# Autodesk Inventor assembly: ROBUSTAv2
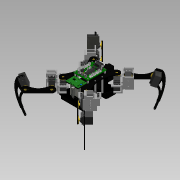
[picture p0: Inventor's stored thumbnail of the model, 180x180]
Saved by Autodesk Inventor 2015 SP1 (Build 190203100, 203)
## iProperties
Created: 2015-01-25
Part Number: ROBUSTAv2
Document SubType Name: Assembly
Designer: Rafi Kurnia Putra
Author: Rafi Kurnia Putra
## Documents named in this file (19)
- D:\Dropbox\krpai berkaki trui 2015\ROBUSTA\MEKANIK\ROBUSTA\Assembly Base.iam
- D:\Dropbox\krpai berkaki trui 2015\ROBUSTA\MEKANIK\ROBUSTA\Base Bawah V2.ipt
- D:\Dropbox\krpai berkaki trui 2015\ROBUSTA\MEKANIK\ROBUSTA\Base Atas V2.ipt
- D:\Dropbox\krpai berkaki trui 2015\ROBUSTA\MEKANIK\ROBUSTA\Spacer 5cm.ipt
- D:\Dropbox\krpai berkaki trui 2015\ROBUSTA\MEKANIK\ROBUSTA\Cover UBEC.ipt
- D:\Dropbox\krpai berkaki trui 2015\ROBUSTA\MEKANIK\ROBUSTA\ssc-32.ipt
- D:\Dropbox\krpai berkaki trui 2015\ROBUSTA\MEKANIK\ROBUSTA\Spacer 1cm.ipt
- D:\Dropbox\krpai berkaki trui 2015\ROBUSTA\MEKANIK\ROBUSTA\servo.ipt
- D:\Dropbox\krpai berkaki trui 2015\ROBUSTA\MEKANIK\ROBUSTA\Horn Servo.ipt
- D:\Dropbox\krpai berkaki trui 2015\ROBUSTA\MEKANIK\ROBUSTA\Femur.ipt
- D:\Dropbox\krpai berkaki trui 2015\ROBUSTA\MEKANIK\ROBUSTA\Bearing Besar.ipt
- D:\Dropbox\krpai berkaki trui 2015\ROBUSTA\MEKANIK\ROBUSTA\Assembly UVTRON.iam
- D:\Dropbox\krpai berkaki trui 2015\ROBUSTA\MEKANIK\ROBUSTA\UVTRON Wall.ipt
- D:\Dropbox\krpai berkaki trui 2015\ROBUSTA\MEKANIK\ROBUSTA\Cover Color Sensor V2.ipt
- D:\Dropbox\krpai berkaki trui 2015\ROBUSTA\MEKANIK\ROBUSTA\2-56 X 0.250 PHS (PHS-02).ipt
- D:\Dropbox\krpai berkaki trui 2015\ROBUSTA\MEKANIK\ROBUSTA\tibia.ipt
- D:\Dropbox\krpai berkaki trui 2015\ROBUSTA\MEKANIK\ROBUSTA\Baterai.ipt
- D:\Dropbox\krpai berkaki trui 2015\ROBUSTA\MEKANIK\ROBUSTA\Braket Servo 2.ipt
- D:\Dropbox\krpai berkaki trui 2015\ROBUSTA\MEKANIK\ROBUSTA\Bracket3.ipt
## Components (67 placed, 18 different names)
1. Base Bawah V2:1 — Mate:1, Mate:2, Mate:3, Mate:4, Mate:5, Mate:6, Mate:7, Mate:8, Mate:13, Mate:14, Mate:15, Mate:169, Mate:170, Mate:171, Mate:203, Mate:204, Mate:205, Mate:311, Angle:18, Flush:2, Flush:3, Angle:19
2. Spacer 5cm:1 — Mate:1, Mate:2, Mate:175, Mate:184, Angle:15, Angle:17, Mate:312
3. Spacer 5cm:2 — Mate:3, Mate:4, Mate:174, Mate:185, Angle:16
4. Spacer 5cm:3 — Mate:5, Mate:6, Mate:172, Angle:16
5. Spacer 5cm:4 — Mate:7, Mate:8, Mate:173, Angle:15
6. Cover UBEC:1 — Mate:13, Mate:14, Mate:15, Insert:7, Insert:8, Mate:314
7. Spacer 1cm:1 — Insert:4, Mate:183, Mate:186
8. Spacer 1cm:2 — Insert:3, Mate:180, Mate:187
9. Spacer 1cm:3 — Mate:181, Mate:188
10. Spacer 1cm:4 — Mate:182, Mate:189
11. ssc-32:1 — Insert:3, Insert:4
12. servo:1 — Mate:28, Mate:29, Mate:290, Mate:291, Mate:292, Angle:13
13. Horn Servo:1 — Mate:28, Mate:29, Mate:152, Mate:153
14. Braket Servo 2:1 — Mate:34, Mate:35, Mate:37, Mate:38, Mate:39, Mate:315, Mate:317
15. Braket Servo 2:2 — Mate:34, Mate:35, Mate:45, Mate:46, Mate:47, Mate:141, Angle:19, Mate:315, Mate:316, Angle:20
16. servo:2 — Mate:37, Mate:38, Mate:39, Mate:40, Mate:41, Mate:42, Mate:318, Mate:319
17. Horn Servo:3 — Mate:40, Mate:41, Mate:42, Mate:150, Mate:151
18. servo:3 — Mate:45, Mate:46, Mate:47, Mate:48, Mate:49
19. Horn Servo:4 — Mate:48, Mate:49, Mate:193, Mate:194
20. servo:4 — Mate:296, Mate:297, Mate:298, Angle:9
21. Horn Servo:5 — Mate:160, Mate:161
22. Braket Servo 2:5 — Mate:325, Mate:327
23. Braket Servo 2:6 — Mate:145, Mate:325, Mate:326, Angle:22
24. servo:5 — Mate:328, Mate:329
25. Horn Servo:6 — Mate:158, Mate:159
26. servo:6 — Angle:7
27. Horn Servo:7 — Mate:191, Mate:196
28. servo:7 — Mate:80, Mate:81, Mate:293, Mate:294, Mate:295, Angle:6
29. Horn Servo:8 — Mate:80, Mate:81, Mate:156, Mate:157
30. Braket Servo 2:4 — Mate:84, Mate:85, Mate:86, Mate:87, Mate:143, Mate:304, Mate:305, 90, Mate:320, Mate:321, Angle:21
31. Braket Servo 2:3 — Mate:84, Mate:85, Mate:86, Mate:92, Mate:93, Mate:94, Mate:320, Mate:322, Mate:323, Mate:324
32. servo:8 — Mate:87, Mate:90, Mate:91, Mate:304, Mate:305
33. Horn Servo:9 — Mate:90, Mate:91, Mate:192, Mate:197
34. servo:9 — Mate:92, Mate:93, Mate:94, Mate:95, Mate:96
35. Horn Servo:10 — Mate:95, Mate:96, Mate:154, Mate:155
36. servo:10 — Mate:299, Mate:300, Mate:301, Angle:12
37. Horn Servo:11 — Mate:164, Mate:165
38. Braket Servo 2:8 — Mate:147, Angle:10, Mate:330, Mate:331, Angle:23
39. Braket Servo 2:7 — Mate:330
40. servo:11
41. Horn Servo:12 — Mate:190, Mate:195
42. servo:12
43. Horn Servo:13 — Mate:162, Mate:163
44. Bearing Besar:1 — Mate:141, Mate:316
45. Bearing Besar:2 — Mate:143, Mate:321
46. Bearing Besar:3 — Mate:145, Mate:326
47. Bearing Besar:4 — Mate:147, Mate:331
48. Femur:1 — Mate:150, Mate:151, Mate:152, Mate:153, Angle:13, Angle:20
49. Femur:2 — Mate:154, Mate:155, Mate:156, Mate:157, Angle:6, Angle:21
50. Femur:3 — Mate:158, Mate:159, Mate:160, Mate:161, Angle:9, Angle:22
51. Femur:4 — Mate:162, Mate:163, Mate:164, Mate:165, Angle:12, Angle:23
52. UVTRON Wall:1 — Mate:169, Mate:170, Mate:171, Tangent:1
53. Base Atas V2:1 — Mate:172, Mate:173, Mate:174, Mate:175, Mate:180, Mate:181, Mate:182, Mate:183, Mate:184, Mate:185, Mate:186, Mate:187, Mate:188, Mate:189, Mate:190, Mate:191, Mate:192, Mate:193, Mate:194, Mate:195, Mate:196, Mate:197, 90, Angle:7, Angle:10, Mate:306, Mate:307, Mate:308, Mate:309, Mate:310
54. Cover Color Sensor V2:1 — Mate:203, Mate:204, Mate:205, Insert:5, Insert:6
55. 2-56 X 0.250 PHS (PHS-02):1 — Insert:6
56. 2-56 X 0.250 PHS (PHS-02):2 — Insert:5
57. 2-56 X 0.250 PHS (PHS-02):3 — Insert:7
58. 2-56 X 0.250 PHS (PHS-02):4 — Insert:8
59. tibia:1 — Mate:290, Mate:291, Mate:292
60. tibia:2 — Mate:296, Mate:297, Mate:298
61. tibia:3 — Mate:299, Mate:300, Mate:301
62. tibia:4 — Mate:293, Mate:294, Mate:295
63. Assembly UVTRON:1 [sub-assembly] — Mate:306, Mate:307, Mate:308, Mate:309, Mate:310
64. Baterai:1 — Mate:311, Angle:17, Mate:312, Tangent:1, Angle:18
65. Bracket3:1 — Mate:317, Mate:318, Mate:319
66. Bracket3:2 — Mate:322, Mate:323, Mate:324
67. Bracket3:3 — Mate:327, Mate:328, Mate:329
## Relationships (180: Mate 155, Angle 16, Insert 6, Flush 2, Tangent 1)
- Mate:1: Base Bawah V2:1 ↔ Spacer 5cm:1
- Mate:2: Base Bawah V2:1 ↔ Spacer 5cm:1
- Mate:3: Base Bawah V2:1 ↔ Spacer 5cm:2
- Mate:4: Base Bawah V2:1 ↔ Spacer 5cm:2
- Mate:5: Base Bawah V2:1 ↔ Spacer 5cm:3
- Mate:6: Base Bawah V2:1 ↔ Spacer 5cm:3
- Mate:7: Base Bawah V2:1 ↔ Spacer 5cm:4
- Mate:8: Base Bawah V2:1 ↔ Spacer 5cm:4
- Mate:13: Base Bawah V2:1 ↔ Cover UBEC:1
- Mate:14: Base Bawah V2:1 ↔ Cover UBEC:1
- Mate:15: Base Bawah V2:1 ↔ Cover UBEC:1
- Insert:3: Spacer 1cm:2 ↔ ssc-32:1
- Insert:4: Spacer 1cm:1 ↔ ssc-32:1
- Mate:28: servo:1 ↔ Horn Servo:1
- Mate:29: servo:1 ↔ Horn Servo:1
- Mate:34: Braket Servo 2:1 ↔ Braket Servo 2:2
- Mate:35: Braket Servo 2:1 ↔ Braket Servo 2:2
- Mate:37: Braket Servo 2:1 ↔ servo:2
- Mate:38: Braket Servo 2:1 ↔ servo:2
- Mate:39: Braket Servo 2:1 ↔ servo:2
- Mate:40: servo:2 ↔ Horn Servo:3
- Mate:41: servo:2 ↔ Horn Servo:3
- Mate:42: servo:2 ↔ Horn Servo:3
- Mate:45: Braket Servo 2:2 ↔ servo:3
- Mate:46: Braket Servo 2:2 ↔ servo:3
- Mate:47: Braket Servo 2:2 ↔ servo:3
- Mate:48: servo:3 ↔ Horn Servo:4
- Mate:49: servo:3 ↔ Horn Servo:4
- [Mate]: servo:4 ↔ Horn Servo:5
- [Mate]: servo:4 ↔ Horn Servo:5
- [Mate]: Braket Servo 2:5 ↔ Braket Servo 2:6
- [Mate]: Braket Servo 2:5 ↔ Braket Servo 2:6
- [Mate]: Braket Servo 2:5 ↔ servo:5
- [Mate]: Braket Servo 2:5 ↔ servo:5
- [Mate]: Braket Servo 2:5 ↔ servo:5
- [Mate]: servo:5 ↔ Horn Servo:6
- [Mate]: servo:5 ↔ Horn Servo:6
- [Mate]: servo:5 ↔ Horn Servo:6
- [Mate]: Braket Servo 2:6 ↔ servo:6
- [Mate]: Braket Servo 2:6 ↔ servo:6
- [Mate]: Braket Servo 2:6 ↔ servo:6
- [Mate]: servo:6 ↔ Horn Servo:7
- [Mate]: servo:6 ↔ Horn Servo:7
- Mate:80: servo:7 ↔ Horn Servo:8
- Mate:81: servo:7 ↔ Horn Servo:8
- Mate:84: Braket Servo 2:4 ↔ Braket Servo 2:3
- Mate:85: Braket Servo 2:4 ↔ Braket Servo 2:3
- Mate:86: Braket Servo 2:4 ↔ Braket Servo 2:3
- Mate:87: Braket Servo 2:4 ↔ servo:8
- Mate:90: servo:8 ↔ Horn Servo:9
- Mate:91: servo:8 ↔ Horn Servo:9
- Mate:92: Braket Servo 2:3 ↔ servo:9
- Mate:93: Braket Servo 2:3 ↔ servo:9
- Mate:94: Braket Servo 2:3 ↔ servo:9
- Mate:95: servo:9 ↔ Horn Servo:10
- Mate:96: servo:9 ↔ Horn Servo:10
- [Mate]: servo:10 ↔ Horn Servo:11
- [Mate]: servo:10 ↔ Horn Servo:11
- [Mate]: Braket Servo 2:8 ↔ Braket Servo 2:7
- [Mate]: Braket Servo 2:8 ↔ Braket Servo 2:7
- [Mate]: Braket Servo 2:8 ↔ servo:11
- [Mate]: Braket Servo 2:8 ↔ servo:11
- [Mate]: Braket Servo 2:8 ↔ servo:11
- [Mate]: servo:11 ↔ Horn Servo:12
- [Mate]: servo:11 ↔ Horn Servo:12
- [Mate]: Braket Servo 2:7 ↔ servo:12
- [Mate]: Braket Servo 2:7 ↔ servo:12
- [Mate]: Braket Servo 2:7 ↔ servo:12
- [Mate]: servo:12 ↔ Horn Servo:13
- [Mate]: servo:12 ↔ Horn Servo:13
- Mate:141: Braket Servo 2:2 ↔ Bearing Besar:1
- Mate:143: Braket Servo 2:4 ↔ Bearing Besar:2
- Mate:145: Braket Servo 2:6 ↔ Bearing Besar:3
- Mate:147: Braket Servo 2:8 ↔ Bearing Besar:4
- Mate:150: Horn Servo:3 ↔ Femur:1
- Mate:151: Horn Servo:3 ↔ Femur:1
- Mate:152: Horn Servo:1 ↔ Femur:1
- Mate:153: Horn Servo:1 ↔ Femur:1
- Mate:154: Horn Servo:10 ↔ Femur:2
- Mate:155: Horn Servo:10 ↔ Femur:2
- Mate:156: Horn Servo:8 ↔ Femur:2
- Mate:157: Horn Servo:8 ↔ Femur:2
- Mate:158: Horn Servo:6 ↔ Femur:3
- Mate:159: Horn Servo:6 ↔ Femur:3
- Mate:160: Horn Servo:5 ↔ Femur:3
- Mate:161: Horn Servo:5 ↔ Femur:3
- Mate:162: Horn Servo:13 ↔ Femur:4
- Mate:163: Horn Servo:13 ↔ Femur:4
- Mate:164: Horn Servo:11 ↔ Femur:4
- Mate:165: Horn Servo:11 ↔ Femur:4
- Mate:169: Base Bawah V2:1 ↔ UVTRON Wall:1
- Mate:170: Base Bawah V2:1 ↔ UVTRON Wall:1
- Mate:171: Base Bawah V2:1 ↔ UVTRON Wall:1
- Mate:172: Spacer 5cm:3 ↔ Base Atas V2:1
- Mate:173: Spacer 5cm:4 ↔ Base Atas V2:1
- Mate:174: Spacer 5cm:2 ↔ Base Atas V2:1
- Mate:175: Spacer 5cm:1 ↔ Base Atas V2:1
- Mate:180: Spacer 1cm:2 ↔ Base Atas V2:1
- Mate:181: Spacer 1cm:3 ↔ Base Atas V2:1
- Mate:182: Spacer 1cm:4 ↔ Base Atas V2:1
- Mate:183: Spacer 1cm:1 ↔ Base Atas V2:1
- Mate:184: Spacer 5cm:1 ↔ Base Atas V2:1
- Mate:185: Spacer 5cm:2 ↔ Base Atas V2:1
- Mate:186: Spacer 1cm:1 ↔ Base Atas V2:1
- Mate:187: Spacer 1cm:2 ↔ Base Atas V2:1
- Mate:188: Spacer 1cm:3 ↔ Base Atas V2:1
- Mate:189: Spacer 1cm:4 ↔ Base Atas V2:1
- Mate:190: Horn Servo:12 ↔ Base Atas V2:1
- Mate:191: Horn Servo:7 ↔ Base Atas V2:1
- Mate:192: Horn Servo:9 ↔ Base Atas V2:1
- Mate:193: Horn Servo:4 ↔ Base Atas V2:1
- Mate:194: Horn Servo:4 ↔ Base Atas V2:1
- Mate:195: Horn Servo:12 ↔ Base Atas V2:1
- Mate:196: Horn Servo:7 ↔ Base Atas V2:1
- Mate:197: Horn Servo:9 ↔ Base Atas V2:1
- Mate:203: Base Bawah V2:1 ↔ Cover Color Sensor V2:1
- Mate:204: Base Bawah V2:1 ↔ Cover Color Sensor V2:1
- Mate:205: Base Bawah V2:1 ↔ Cover Color Sensor V2:1
- Insert:5: Cover Color Sensor V2:1 ↔ 2-56 X 0.250 PHS (PHS-02):2
- Insert:6: Cover Color Sensor V2:1 ↔ 2-56 X 0.250 PHS (PHS-02):1
- Insert:7: Cover UBEC:1 ↔ 2-56 X 0.250 PHS (PHS-02):3
- Insert:8: Cover UBEC:1 ↔ 2-56 X 0.250 PHS (PHS-02):4
- Mate:290: servo:1 ↔ tibia:1
- Mate:291: servo:1 ↔ tibia:1
- Mate:292: servo:1 ↔ tibia:1
- Mate:293: servo:7 ↔ tibia:4
- Mate:294: servo:7 ↔ tibia:4
- Mate:295: servo:7 ↔ tibia:4
- Mate:296: servo:4 ↔ tibia:2
- Mate:297: servo:4 ↔ tibia:2
- Mate:298: servo:4 ↔ tibia:2
- Mate:299: servo:10 ↔ tibia:3
- Mate:300: servo:10 ↔ tibia:3
- Mate:301: servo:10 ↔ tibia:3
- Mate:304: Braket Servo 2:4 ↔ servo:8
- Mate:305: Braket Servo 2:4 ↔ servo:8
- 90 [Angle] (135 deg): Braket Servo 2:4 ↔ Base Atas V2:1
- Angle:6 (111.57 deg): servo:7 ↔ Femur:2
- Angle:7 (135 deg): servo:6 ↔ Base Atas V2:1
- Angle:9 (68.43 deg): servo:4 ↔ Femur:3
- Angle:10 (45 deg): Braket Servo 2:8 ↔ Base Atas V2:1
- Angle:12 (111.57 deg): servo:10 ↔ Femur:4
- Angle:13 (111.57 deg): servo:1 ↔ Femur:1
- Mate:306: Base Atas V2:1 ↔ Assembly UVTRON:1
- Mate:307: Base Atas V2:1 ↔ Assembly UVTRON:1
- Mate:308: Base Atas V2:1 ↔ Assembly UVTRON:1
- Mate:309: Base Atas V2:1 ↔ Assembly UVTRON:1
- Mate:310: Base Atas V2:1 ↔ Assembly UVTRON:1
- Mate:311: Base Bawah V2:1 ↔ Baterai:1
- Angle:15 (0 deg): Spacer 5cm:1 ↔ Spacer 5cm:4
- Angle:16 (0 deg): Spacer 5cm:2 ↔ Spacer 5cm:3
- Angle:17 (0 deg): Spacer 5cm:1 ↔ Baterai:1
- Mate:312 (18.977 mm): Spacer 5cm:1 ↔ Baterai:1
- Tangent:1: UVTRON Wall:1 ↔ Baterai:1
- Angle:18 (0 deg): Base Bawah V2:1 ↔ Baterai:1
- Flush:2: Base Bawah V2:1
- Flush:3: Base Bawah V2:1
- Angle:19 (45 deg): Base Bawah V2:1 ↔ Braket Servo 2:2
- Mate:314 (10 mm): Cover UBEC:1
- Mate:315: Braket Servo 2:1 ↔ Braket Servo 2:2
- Mate:316: Braket Servo 2:2 ↔ Bearing Besar:1
- Angle:20 (0 deg): Braket Servo 2:2 ↔ Femur:1
- Mate:317: Braket Servo 2:1 ↔ Bracket3:1
- Mate:318: servo:2 ↔ Bracket3:1
- Mate:319: servo:2 ↔ Bracket3:1
- Mate:320: Braket Servo 2:4 ↔ Braket Servo 2:3
- Mate:321: Braket Servo 2:4 ↔ Bearing Besar:2
- Angle:21 (0 deg): Braket Servo 2:4 ↔ Femur:2
- Mate:322: Braket Servo 2:3 ↔ Bracket3:2
- Mate:323: Braket Servo 2:3 ↔ Bracket3:2
- Mate:324: Braket Servo 2:3 ↔ Bracket3:2
- Mate:325: Braket Servo 2:5 ↔ Braket Servo 2:6
- Mate:326: Braket Servo 2:6 ↔ Bearing Besar:3
- Angle:22 (0 deg): Braket Servo 2:6 ↔ Femur:3
- Mate:327: Braket Servo 2:5 ↔ Bracket3:3
- Mate:328: servo:5 ↔ Bracket3:3
- Mate:329: servo:5 ↔ Bracket3:3
- Mate:330: Braket Servo 2:8 ↔ Braket Servo 2:7
- Mate:331: Braket Servo 2:8 ↔ Bearing Besar:4
- Angle:23 (0 deg): Braket Servo 2:8 ↔ Femur:4
## Named parameters: d71_d41 = 0 mm, d72_d42 = 0 mm, d75_d50 = 0 mm, d76_d51 = 0 mm, d78_d53 = 0 mm, d79_d54 = 0 mm, d80_d55 = 0 mm, d81_d56 = 0 mm, d82_d57 = 0 mm, d83_d58 = 0 mm, d86_d61 = 0 mm, d87_d62 = 0 mm, d88_d63 = 0 mm, d89_d64 = 0 mm, d90_d65 = 0 mm, d120_d98 = 0 mm, d121_d99 = 0 mm, d124_d102 = 0 mm, d125_d103 = 0 mm, d127_d105 = 0 mm, d128_d106 = 0 mm, d129_d107 = 0 mm, d130_d108 = 0 mm, d131_d109 = 0 mm, d132_d110 = 0 mm, d133_d111 = 0 mm, d134_d112 = 0 mm, d135_d113 = 0 mm, d136_d114 = 0 mm
